# Autodesk Inventor assembly: Hilfsbaugruppe Kantensensor für Zeichnung_explosionsansicht
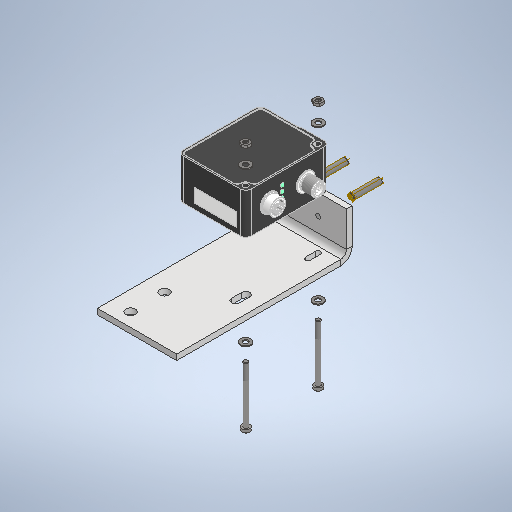
[picture p0: Inventor's stored thumbnail of the model, 512x512]
Saved by Autodesk Inventor 2025.2 (Build 292293000, 293)
## iProperties
Created: 2025-06-24
Part Number: Hilfsbaugruppe Kantensensor für Zeichnung_explosionsansicht
Document SubType Name: Assembly
Designer: Jakob
Author: Jakob
## Documents named in this file (7)
- D:\Useless_Box\CAD-Paspa\Useless Box\Zeichnung_JH\Hilfsbaugruppe Kantensensor für Zeichnung_explosionsansicht.iam
- D:\Useless_Box\CAD-Paspa\Useless Box\Kaufteile\BAUMER_BaumerOXS200117288451\AIS2024\Baumer_OXS200_11728845_1.iam
- D:\Useless_Box\CAD-Paspa\Useless Box\Eigene Bauteile\ER_Halterung_Kantensensor.ipt
- D:\Useless_Box\CAD-Paspa\Useless Box\Standart Bauteile\DIN EN ISO 4026 - M5 x 25.ipt
- D:\Useless_Box\CAD-Paspa\Useless Box\Standart Bauteile\DIN 6912 - M4 x 50.ipt
- D:\Useless_Box\CAD-Paspa\Useless Box\Standart Bauteile\DIN EN ISO 4036 - M4.ipt
- D:\Useless_Box\CAD-Paspa\Useless Box\Standart Bauteile\DIN 125 - A 4,3.ipt
## Components (12 placed, 6 different names)
1. Baumer_OXS200_11728845_1:1 [sub-assembly] — Passend:1, Passend:2, Fluchtend:1, Passend:3, Fluchtend:3, Passend:8, Passend:10, Passend:11, Passend:12
2. ER_Halterung_Kantensensor:1 — Passend:3, Fluchtend:3, Passend:4, Passend:5
3. DIN EN ISO 4026 - M5 x 25:1 — Passend:4, Fluchtend:8
4. DIN EN ISO 4026 - M5 x 25:2 — Passend:5, Fluchtend:8
5. DIN 6912 - M4 x 50:1 — Passend:11, Passend:16, Passend:20, Fluchtend:7
6. DIN 6912 - M4 x 50:2 — Passend:12, Passend:17, Passend:21, Fluchtend:7
7. DIN EN ISO 4036 - M4:1 — Passend:20, Fluchtend:4
8. DIN EN ISO 4036 - M4:2 — Passend:21, Fluchtend:4
9. DIN 125 - A 4,3:1 — Passend:16, Fluchtend:5
10. DIN 125 - A 4,3:2 — Passend:17, Fluchtend:5
11. DIN 125 - A 4,3:3 — Passend:8, Fluchtend:6
12. DIN 125 - A 4,3:4 — Passend:10, Fluchtend:6
## Relationships (20: Mate 13, Flush 7)
- Passend:1 [Mate]: Baumer_OXS200_11728845_1:1
- Passend:2 [Mate]: Baumer_OXS200_11728845_1:1
- Fluchtend:1 [Flush]: Baumer_OXS200_11728845_1:1
- Passend:3 [Mate] (5 mm): Baumer_OXS200_11728845_1:1 ↔ ER_Halterung_Kantensensor:1
- Fluchtend:3 [Flush]: Baumer_OXS200_11728845_1:1 ↔ ER_Halterung_Kantensensor:1
- Passend:4 [Mate]: ER_Halterung_Kantensensor:1 ↔ DIN EN ISO 4026 - M5 x 25:1
- Passend:5 [Mate]: ER_Halterung_Kantensensor:1 ↔ DIN EN ISO 4026 - M5 x 25:2
- Passend:8 [Mate]: Baumer_OXS200_11728845_1:1 ↔ DIN 125 - A 4,3:3
- Passend:10 [Mate]: Baumer_OXS200_11728845_1:1 ↔ DIN 125 - A 4,3:4
- Passend:11 [Mate]: Baumer_OXS200_11728845_1:1 ↔ DIN 6912 - M4 x 50:1
- Passend:12 [Mate]: Baumer_OXS200_11728845_1:1 ↔ DIN 6912 - M4 x 50:2
- Passend:16 [Mate]: DIN 6912 - M4 x 50:1 ↔ DIN 125 - A 4,3:1
- Passend:17 [Mate]: DIN 6912 - M4 x 50:2 ↔ DIN 125 - A 4,3:2
- Passend:20 [Mate]: DIN 6912 - M4 x 50:1 ↔ DIN EN ISO 4036 - M4:1
- Passend:21 [Mate]: DIN 6912 - M4 x 50:2 ↔ DIN EN ISO 4036 - M4:2
- Fluchtend:4 [Flush]: DIN EN ISO 4036 - M4:1 ↔ DIN EN ISO 4036 - M4:2
- Fluchtend:5 [Flush]: DIN 125 - A 4,3:1 ↔ DIN 125 - A 4,3:2
- Fluchtend:6 [Flush]: DIN 125 - A 4,3:3 ↔ DIN 125 - A 4,3:4
- Fluchtend:7 [Flush]: DIN 6912 - M4 x 50:1 ↔ DIN 6912 - M4 x 50:2
- Fluchtend:8 [Flush]: DIN EN ISO 4026 - M5 x 25:1 ↔ DIN EN ISO 4026 - M5 x 25:2
